# Autodesk Inventor assembly: ExampleJoint
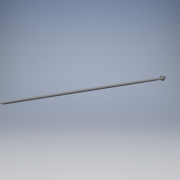
[picture p0: Inventor's stored thumbnail of the model, 180x180]
Saved by Autodesk Inventor 2017.2 (Build 212233000, 233)
## iProperties
Created: 2018-01-21
Part Number: ExampleJoint
Document SubType Name: Assembly
Designer: Vatsal Varma
Author: Vatsal Varma
## Documents named in this file (4)
- C:\Users\Vatsal Varma\Idea\Design & Modeling\InventorProjects\Animatronics\ExampleJoint.iam
- C:\Users\Vatsal Varma\Idea\Design & Modeling\InventorProjects\Animatronics\Ball.ipt
- C:\Users\Vatsal Varma\Idea\Design & Modeling\InventorProjects\Animatronics\Socket.ipt
- C:\Users\Vatsal Varma\Idea\Design & Modeling\InventorProjects\Animatronics\Bone-25cm.ipt
## Components (3 placed, 3 different names)
1. Socket:1 — Ball:1
2. Ball:1 — Ball:1, Insert:1
3. Bone-25cm:1 — Insert:1
## Relationships (2: BallJoint 1, Insert 1)
- Ball:1: Socket:1 ↔ Ball:1
- Insert:1: Ball:1 ↔ Bone-25cm:1
